# Autodesk Inventor assembly: Eslabon3
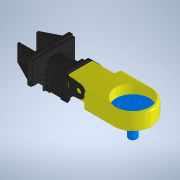
[picture p0: Inventor's stored thumbnail of the model, 180x180]
Saved by Autodesk Inventor 2021 (Build 250183000, 183)
## iProperties
Created: 2022-04-22
Part Number: Eslabon3
Document SubType Name: Assembly
Designer: Alcatraz
Author: Alcatraz
## Documents named in this file (4)
- F:\Tesis\TESIS\Matlab\Pruebas\Prueba3_Simulacion1\Eslabon3.iam
- F:\Tesis\TESIS\Eslabon_Gripper_parametrizado_MPlano_2.ipt
- F:\Tesis\TESIS\GRIPPER_M.iam
- F:\Tesis\TESIS\Eje_3_parametrizado.ipt
## Components (3 placed, 3 different names)
1. Eslabon_Gripper_parametrizado_MPlano_2:1 — Coincidencia:1, Coincidencia:2, Coincidencia:3, Coincidencia:4, Coincidencia:5, Coincidencia:6
2. GRIPPER_M:1 [sub-assembly] — Coincidencia:1, Coincidencia:2, Coincidencia:3
3. Eje_3_parametrizado:1 — Coincidencia:4, Coincidencia:5, Coincidencia:6
## Relationships (6: Mate 6)
- Coincidencia:1 [Mate]: Eslabon_Gripper_parametrizado_MPlano_2:1 ↔ GRIPPER_M:1
- Coincidencia:2 [Mate]: Eslabon_Gripper_parametrizado_MPlano_2:1 ↔ GRIPPER_M:1
- Coincidencia:3 [Mate]: Eslabon_Gripper_parametrizado_MPlano_2:1 ↔ GRIPPER_M:1
- Coincidencia:4 [Mate]: Eslabon_Gripper_parametrizado_MPlano_2:1 ↔ Eje_3_parametrizado:1
- Coincidencia:5 [Mate]: Eslabon_Gripper_parametrizado_MPlano_2:1 ↔ Eje_3_parametrizado:1
- Coincidencia:6 [Mate]: Eslabon_Gripper_parametrizado_MPlano_2:1 ↔ Eje_3_parametrizado:1
